# Autodesk Inventor assembly: каркас с уголками
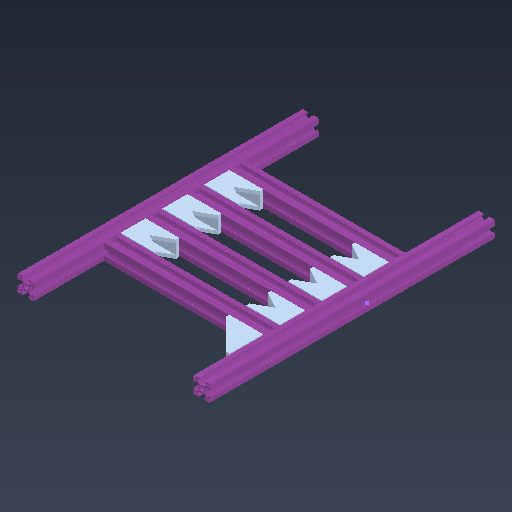
[picture p0: Inventor's stored thumbnail of the model, 512x512]
Saved by Autodesk Inventor 2025 (Build 290162000, 162)
## iProperties
Created: 2025-01-29
Part Number: каркас с уголками
Document SubType Name: Assembly
Designer: GameHD
Author: GameHD
## Documents named in this file (5)
- C:\Users\GameHD\Desktop\phantom 16950\каркас с уголками.iam
- C:\Users\GameHD\Desktop\phantom 16950\профиль каркас.ipt
- C:\Users\GameHD\Desktop\phantom 16950\профиль каркас паралельно.ipt
- C:\Users\GameHD\Desktop\phantom 16950\хвост распорка\хвост распорка.ipt
- C:\Users\GameHD\Desktop\phantom 16950\Уголок (11)\Уголок (11).ipt
## Components (13 placed, 4 different names)
1. профиль каркас:1
2. профиль каркас паралельно:1
3. профиль каркас паралельно:2
4. профиль каркас паралельно:3
5. профиль каркас паралельно:4
6. профиль каркас:2
7. хвост распорка:1
8. Уголок (11):1
9. хвост распорка:2
10. хвост распорка:3
11. хвост распорка:4
12. хвост распорка:5
13. хвост распорка:6
## Relationships (38: Mate 32, Flush 6)
- [Mate]: профиль каркас:1 ↔ профиль каркас паралельно:1
- [Flush]: профиль каркас:1 ↔ профиль каркас паралельно:1
- [Mate]: профиль каркас:1 ↔ профиль каркас паралельно:2
- [Flush]: профиль каркас:1 ↔ профиль каркас паралельно:2
- [Flush]: профиль каркас:1 ↔ профиль каркас паралельно:4
- [Mate]: профиль каркас:1 ↔ профиль каркас паралельно:4
- [Flush]: профиль каркас:1 ↔ профиль каркас паралельно:3
- [Mate]: профиль каркас:1 ↔ профиль каркас паралельно:3
- [Mate]: профиль каркас паралельно:1 ↔ профиль каркас:2
- [Flush]: профиль каркас:1 ↔ профиль каркас:2
- [Flush]: профиль каркас паралельно:3 ↔ профиль каркас:2
- [Mate]: профиль каркас паралельно:4 ↔ хвост распорка:1
- [Mate]: профиль каркас:1 ↔ хвост распорка:1
- [Mate]: профиль каркас паралельно:4 ↔ хвост распорка:1
- [Mate]: профиль каркас паралельно:1 ↔ хвост распорка:1
- [Mate]: профиль каркас паралельно:2 ↔ хвост распорка:2
- [Mate]: профиль каркас паралельно:1 ↔ хвост распорка:2
- [Mate]: профиль каркас:1 ↔ хвост распорка:2
- [Mate]: профиль каркас паралельно:1 ↔ хвост распорка:2
- [Mate]: профиль каркас паралельно:4 ↔ хвост распорка:3
- [Mate]: профиль каркас паралельно:3 ↔ хвост распорка:3
- [Mate]: профиль каркас:1 ↔ хвост распорка:3
- [Mate]: профиль каркас паралельно:3 ↔ хвост распорка:3
- [Mate]: профиль каркас паралельно:3 ↔ Уголок (11):1
- [Mate]: профиль каркас:2 ↔ Уголок (11):1
- [Mate]: профиль каркас:2 ↔ Уголок (11):1
- [Mate]: профиль каркас:2 ↔ хвост распорка:4
- [Mate]: профиль каркас паралельно:4 ↔ хвост распорка:4
- [Mate]: профиль каркас паралельно:1 ↔ хвост распорка:4
- [Mate]: профиль каркас паралельно:1 ↔ хвост распорка:4
- [Mate]: профиль каркас паралельно:2 ↔ хвост распорка:5
- [Mate]: профиль каркас:2 ↔ хвост распорка:5
- [Mate]: профиль каркас паралельно:1 ↔ хвост распорка:5
- [Mate]: профиль каркас паралельно:2 ↔ хвост распорка:5
- [Mate]: профиль каркас паралельно:4 ↔ хвост распорка:6
- [Mate]: профиль каркас:2 ↔ хвост распорка:6
- [Mate]: профиль каркас паралельно:3 ↔ хвост распорка:6
- [Mate]: профиль каркас паралельно:3 ↔ хвост распорка:6
